# Autodesk Inventor assembly: New Final Assembly
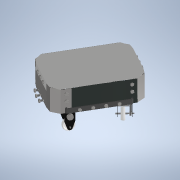
[picture p0: Inventor's stored thumbnail of the model, 180x180]
Saved by Autodesk Inventor 2020 (Build 240168000, 168)
## iProperties
Created: 2022-07-18
Part Number: New Final Assembly
Document SubType Name: Assembly
Designer: karimi2
Author: karimi2
## Documents named in this file (4)
- C:\Users\karimi2\Documents\PROJECT\src\New Final Assembly.iam
- C:\Users\karimi2\Documents\PROJECT\src\New redesign Assembly.iam
- C:\Users\karimi2\Documents\PROJECT\src\Latest Assembly.iam
- C:\Users\karimi2\Documents\Inventor\Content Center Files\R2020\en-US\CNS 4308 - AB\CNS 4308 - M8 x 16AB.ipt
## Components (34 placed, 3 different names)
1. New redesign Assembly:1 [sub-assembly] — Mate:1, Mate:2, Mate:3, Mate:4, Mate:5, Mate:6, Mate:7, Mate:8, Mate:9, Mate:10, Mate:11, Mate:15, Mate:16, Mate:17, Mate:19, Mate:20, Mate:25, Mate:26, Mate:27, Mate:31, Mate:32, Mate:33, Mate:34, Mate:35, Mate:40, Mate:41, Mate:43, Mate:44, Mate:45, Mate:46, Mate:47, Mate:48, Mate:49, Mate:50, Mate:51, Mate:52, Mate:53, Mate:54, Mate:55, Mate:56, Mate:57, Mate:58, Mate:59, Mate:60, Mate:61, Mate:62, Mate:63
2. Latest Assembly:1 [sub-assembly] — Mate:1, Mate:2, Mate:3, Mate:12, Mate:13, Mate:14, Mate:21, Mate:22, Mate:24, Mate:28, Mate:29, Mate:30, Mate:36, Mate:37, Mate:38, Mate:39, Mate:42, Mate:64
3. CNS 4308 - AB M8 x 16:1 — Mate:10, Mate:49
4. CNS 4308 - AB M8 x 16:2 — Mate:9, Mate:50
5. CNS 4308 - AB M8 x 16:3 — Mate:4, Mate:55
6. CNS 4308 - AB M8 x 16:4 — Mate:7, Mate:52
7. CNS 4308 - AB M8 x 16:5 — Mate:5, Mate:54
8. CNS 4308 - AB M8 x 16:6 — Mate:6, Mate:53
9. CNS 4308 - AB M8 x 16:7 — Mate:8, Mate:51
10. CNS 4308 - AB M8 x 16:8 — Mate:15, Mate:62
11. CNS 4308 - AB M8 x 16:9 — Mate:11, Mate:63
12. CNS 4308 - AB M8 x 16:10 — Mate:12
13. CNS 4308 - AB M8 x 16:11 — Mate:29, Mate:48
14. CNS 4308 - AB M8 x 16:12 — Mate:13
15. CNS 4308 - AB M8 x 16:13 — Mate:14
16. CNS 4308 - AB M8 x 16:14 — Mate:16, Mate:61
17. CNS 4308 - AB M8 x 16:15 — Mate:20, Mate:35
18. CNS 4308 - AB M8 x 16:16 — Mate:33, Mate:56
19. CNS 4308 - AB M8 x 16:17 — Mate:21, Mate:38
20. CNS 4308 - AB M8 x 16:18 — Mate:19, Mate:34
21. CNS 4308 - AB M8 x 16:19 — Mate:31, Mate:58
22. CNS 4308 - AB M8 x 16:20 — Mate:30, Mate:46
23. CNS 4308 - AB M8 x 16:21 — Mate:24, Mate:37
24. CNS 4308 - AB M8 x 16:22 — Mate:22
25. CNS 4308 - AB M8 x 16:24 — Mate:32, Mate:57
26. CNS 4308 - AB M8 x 16:25 — Mate:17
27. CNS 4308 - AB M8 x 16:27 — Mate:27, Mate:45
28. CNS 4308 - AB M8 x 16:28 — Mate:28, Mate:47
29. CNS 4308 - AB M8 x 16:29 — Mate:40, Mate:59
30. CNS 4308 - AB M8 x 16:30 — Mate:25, Mate:43
31. CNS 4308 - AB M8 x 16:31 — Mate:26, Mate:44
32. CNS 4308 - AB M8 x 16:32 — Mate:36, Mate:39
33. CNS 4308 - AB M8 x 16:33 — Mate:41, Mate:60
34. CNS 4308 - AB M8 x 16:34 — Mate:42, Mate:64
## Relationships (62: Mate 62)
- Mate:1: New redesign Assembly:1 ↔ Latest Assembly:1
- Mate:2: New redesign Assembly:1 ↔ Latest Assembly:1
- Mate:3: New redesign Assembly:1 ↔ Latest Assembly:1
- Mate:4: New redesign Assembly:1 ↔ CNS 4308 - AB M8 x 16:3
- Mate:5: New redesign Assembly:1 ↔ CNS 4308 - AB M8 x 16:5
- Mate:6: New redesign Assembly:1 ↔ CNS 4308 - AB M8 x 16:6
- Mate:7: New redesign Assembly:1 ↔ CNS 4308 - AB M8 x 16:4
- Mate:8: New redesign Assembly:1 ↔ CNS 4308 - AB M8 x 16:7
- Mate:9: New redesign Assembly:1 ↔ CNS 4308 - AB M8 x 16:2
- Mate:10: New redesign Assembly:1 ↔ CNS 4308 - AB M8 x 16:1
- Mate:11: New redesign Assembly:1 ↔ CNS 4308 - AB M8 x 16:9
- Mate:12: Latest Assembly:1 ↔ CNS 4308 - AB M8 x 16:10
- Mate:13: Latest Assembly:1 ↔ CNS 4308 - AB M8 x 16:12
- Mate:14: Latest Assembly:1 ↔ CNS 4308 - AB M8 x 16:13
- Mate:15: New redesign Assembly:1 ↔ CNS 4308 - AB M8 x 16:8
- Mate:16: New redesign Assembly:1 ↔ CNS 4308 - AB M8 x 16:14
- Mate:17: New redesign Assembly:1 ↔ CNS 4308 - AB M8 x 16:25
- Mate:19: New redesign Assembly:1 ↔ CNS 4308 - AB M8 x 16:18
- Mate:20: New redesign Assembly:1 ↔ CNS 4308 - AB M8 x 16:15
- Mate:21: Latest Assembly:1 ↔ CNS 4308 - AB M8 x 16:17
- Mate:22: Latest Assembly:1 ↔ CNS 4308 - AB M8 x 16:22
- Mate:24: Latest Assembly:1 ↔ CNS 4308 - AB M8 x 16:21
- Mate:25: New redesign Assembly:1 ↔ CNS 4308 - AB M8 x 16:30
- Mate:26: New redesign Assembly:1 ↔ CNS 4308 - AB M8 x 16:31
- Mate:27: New redesign Assembly:1 ↔ CNS 4308 - AB M8 x 16:27
- Mate:28: Latest Assembly:1 ↔ CNS 4308 - AB M8 x 16:28
- Mate:29: Latest Assembly:1 ↔ CNS 4308 - AB M8 x 16:11
- Mate:30: Latest Assembly:1 ↔ CNS 4308 - AB M8 x 16:20
- Mate:31: New redesign Assembly:1 ↔ CNS 4308 - AB M8 x 16:19
- Mate:32: New redesign Assembly:1 ↔ CNS 4308 - AB M8 x 16:24
- Mate:33: New redesign Assembly:1 ↔ CNS 4308 - AB M8 x 16:16
- Mate:34: New redesign Assembly:1 ↔ CNS 4308 - AB M8 x 16:18
- Mate:35: New redesign Assembly:1 ↔ CNS 4308 - AB M8 x 16:15
- Mate:36: Latest Assembly:1 ↔ CNS 4308 - AB M8 x 16:32
- Mate:37: Latest Assembly:1 ↔ CNS 4308 - AB M8 x 16:21
- Mate:38: Latest Assembly:1 ↔ CNS 4308 - AB M8 x 16:17
- Mate:39: Latest Assembly:1 ↔ CNS 4308 - AB M8 x 16:32
- Mate:40: New redesign Assembly:1 ↔ CNS 4308 - AB M8 x 16:29
- Mate:41: New redesign Assembly:1 ↔ CNS 4308 - AB M8 x 16:33
- Mate:42: Latest Assembly:1 ↔ CNS 4308 - AB M8 x 16:34
- Mate:43: New redesign Assembly:1 ↔ CNS 4308 - AB M8 x 16:30
- Mate:44: New redesign Assembly:1 ↔ CNS 4308 - AB M8 x 16:31
- Mate:45: New redesign Assembly:1 ↔ CNS 4308 - AB M8 x 16:27
- Mate:46: New redesign Assembly:1 ↔ CNS 4308 - AB M8 x 16:20
- Mate:47: New redesign Assembly:1 ↔ CNS 4308 - AB M8 x 16:28
- Mate:48: New redesign Assembly:1 ↔ CNS 4308 - AB M8 x 16:11
- Mate:49: New redesign Assembly:1 ↔ CNS 4308 - AB M8 x 16:1
- Mate:50: New redesign Assembly:1 ↔ CNS 4308 - AB M8 x 16:2
- Mate:51: New redesign Assembly:1 ↔ CNS 4308 - AB M8 x 16:7
- Mate:52: New redesign Assembly:1 ↔ CNS 4308 - AB M8 x 16:4
- Mate:53: New redesign Assembly:1 ↔ CNS 4308 - AB M8 x 16:6
- Mate:54: New redesign Assembly:1 ↔ CNS 4308 - AB M8 x 16:5
- Mate:55: New redesign Assembly:1 ↔ CNS 4308 - AB M8 x 16:3
- Mate:56: New redesign Assembly:1 ↔ CNS 4308 - AB M8 x 16:16
- Mate:57: New redesign Assembly:1 ↔ CNS 4308 - AB M8 x 16:24
- Mate:58: New redesign Assembly:1 ↔ CNS 4308 - AB M8 x 16:19
- Mate:59: New redesign Assembly:1 ↔ CNS 4308 - AB M8 x 16:29
- Mate:60: New redesign Assembly:1 ↔ CNS 4308 - AB M8 x 16:33
- Mate:61: New redesign Assembly:1 ↔ CNS 4308 - AB M8 x 16:14
- Mate:62: New redesign Assembly:1 ↔ CNS 4308 - AB M8 x 16:8
- Mate:63: New redesign Assembly:1 ↔ CNS 4308 - AB M8 x 16:9
- Mate:64: Latest Assembly:1 ↔ CNS 4308 - AB M8 x 16:34
